# Autodesk Inventor assembly: Tensionador-3-Cabos
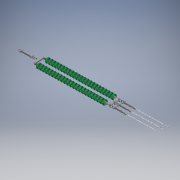
[picture p0: Inventor's stored thumbnail of the model, 180x180]
Saved by Autodesk Inventor 2018 (Build 220112000, 112)
## iProperties
Created: 2021-04-28
Part Number: Tensionador-3-Cabos
Document SubType Name: Assembly
Designer: l01767
Author: l01767
## Documents named in this file (10)
- F:\Projetos\TAESA\Modelo 3D - Tensionadores e Suspensão\Tensionador\Tensionador-3-Cabos.iam
- F:\Projetos\TAESA\Modelo 3D - Tensionadores e Suspensão\Tensionador\gpghmb32.iam
- F:\Projetos\TAESA\Modelo 3D - Tensionadores e Suspensão\Tensionador\Link_Principal.ipt
- F:\Projetos\TAESA\Modelo 3D - Tensionadores e Suspensão\Tensionador\Espacador_Delta.ipt
- F:\Projetos\TAESA\Modelo 3D - Tensionadores e Suspensão\Tensionador\Clevis-Bola_Curto.ipt
- F:\Projetos\TAESA\Modelo 3D - Tensionadores e Suspensão\Tensionador\Bolted Connection1.iam
- F:\Projetos\TAESA\Modelo 3D - Tensionadores e Suspensão\Tensionador\U300B.iam
- F:\Projetos\TAESA\Modelo 3D - Tensionadores e Suspensão\Tensionador\Clevis-Socket.iam
- F:\Projetos\TAESA\Modelo 3D - Tensionadores e Suspensão\Tensionador\Balancim_Duplicador.ipt
- F:\Projetos\TAESA\Modelo 3D - Tensionadores e Suspensão\Tensionador\OPGW Tension set.iam
## Components (67 placed, 9 different names)
1. gpghmb32:1 [sub-assembly] — Mate:1, Mate:2, Flush:1, Mate:3, Mate:4, Mate:6
2. gpghmb32:2 [sub-assembly] — Mate:5, Mate:7, Flush:2, Flush:11, Flush:10, Tangent:1
3. Link_Principal:1 — Mate:1, Mate:4, Mate:5, Mate:6, Mate:7, Flush:2
4. gpghmb32:3 [sub-assembly] — Flush:11, Flush:10, Tangent:1, Mate:8, Mate:9, Mate:10
5. Espacador_Delta:1 — Mate:8, Mate:9, Mate:10, Mate:11, Angle:1, Mate:12
6. Clevis-Socket:1 [sub-assembly] — Mate:23, Mate:24, Mate:30
7. Clevis-Socket:3 [sub-assembly] — Mate:27, Mate:28, Mate:29
8. Balancim_Duplicador:1 — Mate:29, Mate:30, Mate:32, Mate:33, Flush:12, Angle:10, Cylindrical:1, Cylindrical:2, Mate:46, Mate:47, Angle:11, Angle:12
9. gpghmb32:4 [sub-assembly] — Mate:32, Mate:33, Flush:12, Flush:13, Flush:14, Tangent:2
10. gpghmb32:5 [sub-assembly] — Flush:13, Flush:14, Tangent:2, Mate:45
11. OPGW Tension set:1 [sub-assembly] — Mate:45, Angle:10
12. gpghmb32:6 [sub-assembly] — Cylindrical:1, Mate:47, Angle:11, Flush:20, Flush:22, Tangent:4
13. gpghmb32:7 [sub-assembly] — Cylindrical:2, Mate:46, Angle:12, Flush:19, Flush:21, Tangent:3
14. gpghmb32:8 [sub-assembly] — Flush:19, Flush:21, Tangent:3, Mate:48, Flush:53
15. gpghmb32:9 [sub-assembly] — Flush:20, Flush:22, Tangent:4, Mate:49, Flush:52
16. OPGW Tension set:2 [sub-assembly] — Mate:49, Flush:52
17. OPGW Tension set:3 [sub-assembly] — Mate:48, Flush:53
18. Clevis-Bola_Curto:1 — Mate:11, Angle:1, Mate:12, Mate:13, Mate:14, Mate:15, Mate:16, Angle:2
19. Bolted Connection:1 [sub-assembly] — Mate:13, Mate:14
20. Clevis-Bola_Curto:2
21. Bolted Connection:2 [sub-assembly]
22. U300B:1 [sub-assembly] — Mate:15, Mate:16, Angle:2
23. U300B:2 [sub-assembly]
24. U300B:3 [sub-assembly]
25. U300B:4 [sub-assembly]
26. U300B:5 [sub-assembly]
27. U300B:6 [sub-assembly]
28. U300B:7 [sub-assembly]
29. U300B:8 [sub-assembly]
30. U300B:9 [sub-assembly]
31. U300B:10 [sub-assembly]
32. U300B:11 [sub-assembly]
33. U300B:12 [sub-assembly]
34. U300B:13 [sub-assembly]
35. U300B:14 [sub-assembly]
36. U300B:15 [sub-assembly]
37. U300B:16 [sub-assembly]
38. U300B:17 [sub-assembly]
39. U300B:18 [sub-assembly]
40. U300B:19 [sub-assembly]
41. U300B:20 [sub-assembly]
42. U300B:21 [sub-assembly]
43. U300B:22 [sub-assembly]
44. U300B:23 [sub-assembly] — Mate:23, Mate:24
45. U300B:24 [sub-assembly]
46. U300B:25 [sub-assembly]
47. U300B:26 [sub-assembly]
48. U300B:27 [sub-assembly]
49. U300B:28 [sub-assembly]
50. U300B:29 [sub-assembly]
51. U300B:30 [sub-assembly]
52. U300B:31 [sub-assembly]
53. U300B:32 [sub-assembly]
54. U300B:33 [sub-assembly]
55. U300B:34 [sub-assembly]
56. U300B:35 [sub-assembly]
57. U300B:36 [sub-assembly]
58. U300B:37 [sub-assembly]
59. U300B:38 [sub-assembly]
60. U300B:39 [sub-assembly]
61. U300B:40 [sub-assembly]
62. U300B:41 [sub-assembly]
63. U300B:42 [sub-assembly]
64. U300B:43 [sub-assembly]
65. U300B:44 [sub-assembly]
66. U300B:45 [sub-assembly]
67. U300B:46 [sub-assembly] — Mate:27, Mate:28
## Component patterns: (2 elements, first: Clevis-Bola_Curto:1 + Bolted Connection:1), (23 elements, first: U300B:1), Component Pattern 1:2 (23 elements)
## Relationships (53: Mate 29, Flush 13, Angle 5, Tangent 4, CylindricalJoint 2)
- Mate:1: gpghmb32:1 ↔ Link_Principal:1
- Mate:2: gpghmb32:1
- Flush:1: gpghmb32:1
- Mate:3: gpghmb32:1
- Mate:4: gpghmb32:1 ↔ Link_Principal:1
- Mate:5: gpghmb32:2 ↔ Link_Principal:1
- Mate:6: gpghmb32:1 ↔ Link_Principal:1
- Mate:7: gpghmb32:2 ↔ Link_Principal:1
- Flush:2: gpghmb32:2 ↔ Link_Principal:1
- Flush:11: gpghmb32:2 ↔ gpghmb32:3
- Flush:10: gpghmb32:2 ↔ gpghmb32:3
- Tangent:1: gpghmb32:2 ↔ gpghmb32:3
- Mate:8: gpghmb32:3 ↔ Espacador_Delta:1
- Mate:9: gpghmb32:3 ↔ Espacador_Delta:1
- Mate:10: gpghmb32:3 ↔ Espacador_Delta:1
- Mate:11: Espacador_Delta:1 ↔ Clevis-Bola_Curto:1
- Angle:1 (180 deg): Espacador_Delta:1 ↔ Clevis-Bola_Curto:1
- Mate:12: Espacador_Delta:1 ↔ Clevis-Bola_Curto:1
- Mate:13: Clevis-Bola_Curto:1 ↔ Bolted Connection:1
- Mate:14: Clevis-Bola_Curto:1 ↔ Bolted Connection:1
- Mate:15: Clevis-Bola_Curto:1 ↔ U300B:1
- Mate:16 (5 mm): Clevis-Bola_Curto:1 ↔ U300B:1
- Angle:2 (0 deg): Clevis-Bola_Curto:1 ↔ U300B:1
- Mate:23: Clevis-Socket:1 ↔ U300B:23
- Mate:24 (15 mm): Clevis-Socket:1 ↔ U300B:23
- Mate:27: Clevis-Socket:3 ↔ U300B:46
- Mate:28 (15 mm): Clevis-Socket:3 ↔ U300B:46
- Mate:29: Clevis-Socket:3 ↔ Balancim_Duplicador:1
- Mate:30: Clevis-Socket:1 ↔ Balancim_Duplicador:1
- Mate:32: Balancim_Duplicador:1 ↔ gpghmb32:4
- Mate:33: Balancim_Duplicador:1 ↔ gpghmb32:4
- Flush:12: Balancim_Duplicador:1 ↔ gpghmb32:4
- Flush:13: gpghmb32:4 ↔ gpghmb32:5
- Flush:14: gpghmb32:4 ↔ gpghmb32:5
- Tangent:2: gpghmb32:4 ↔ gpghmb32:5
- Mate:45: gpghmb32:5 ↔ OPGW Tension set:1
- Angle:10 (0 deg): Balancim_Duplicador:1 ↔ OPGW Tension set:1
- Cylindrical:1: Balancim_Duplicador:1 ↔ gpghmb32:6
- Cylindrical:2: Balancim_Duplicador:1 ↔ gpghmb32:7
- Mate:46: Balancim_Duplicador:1 ↔ gpghmb32:7
- Mate:47: Balancim_Duplicador:1 ↔ gpghmb32:6
- Angle:11 (0 deg): Balancim_Duplicador:1 ↔ gpghmb32:6
- Angle:12 (0 deg): Balancim_Duplicador:1 ↔ gpghmb32:7
- Flush:19: gpghmb32:7 ↔ gpghmb32:8
- Flush:20: gpghmb32:6 ↔ gpghmb32:9
- Flush:21: gpghmb32:7 ↔ gpghmb32:8
- Flush:22: gpghmb32:6 ↔ gpghmb32:9
- Tangent:3: gpghmb32:7 ↔ gpghmb32:8
- Tangent:4: gpghmb32:6 ↔ gpghmb32:9
- Mate:48: gpghmb32:8 ↔ OPGW Tension set:3
- Mate:49: gpghmb32:9 ↔ OPGW Tension set:2
- Flush:53: gpghmb32:8 ↔ OPGW Tension set:3
- Flush:52: gpghmb32:9 ↔ OPGW Tension set:2
